# Autodesk Inventor assembly: still pipe
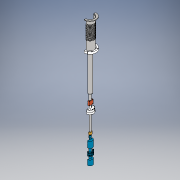
[picture p0: Inventor's stored thumbnail of the model, 180x180]
Saved by Autodesk Inventor 2018 (Build 220112000, 112)
## iProperties
Created: 2019-01-14
Part Number: still pipe
Document SubType Name: Assembly
Designer: Admin
Author: Admin
## Documents named in this file (11)
- C:\Users\Admin\Documents\Cryostat\CAD\still pipe.iam
- C:\Users\Admin\Documents\Cryostat\CAD\KF50 bellows.ipt
- C:\Users\Admin\Documents\Cryostat\CAD\universal connector.ipt
- C:\Users\Admin\Documents\Cryostat\CAD\1in ss pipe.ipt
- C:\Users\Admin\Documents\Cryostat\CAD\adapter.ipt
- C:\Users\Admin\Documents\Cryostat\CAD\heatsink.ipt
- C:\Users\Admin\Documents\Cryostat\CAD\brassbushing2.ipt
- C:\Users\Admin\Documents\Cryostat\CAD\minifridge.ipt
- C:\Users\Admin\Documents\Cryostat\CAD\universal connector male.ipt
- C:\Users\Admin\Documents\Cryostat\CAD\ss pipe for still.ipt
- C:\Users\Admin\Documents\Cryostat\CAD\fridge bushing.ipt
## Components (10 placed, 10 different names)
1. KF50 bellows:1 — Mate:16, Flush:2
2. universal connector:1 — Mate:24, Mate:26, Mate:27, Mate:28, Mate:36
3. 1in ss pipe:3 — Mate:15, Flush:1, Mate:17, Mate:31, Mate:32
4. adapter:1 — Mate:15, Flush:1, Mate:16, Flush:2, Mate:19, Mate:34, Mate:35
5. heatsink:1 — Mate:17, Mate:19, Mate:34, Mate:35
6. brassbushing2:1 — Mate:24, Mate:31, Mate:32, Mate:36
7. minifridge:1 — Mate:41, Mate:42
8. universal connector male:1 — Mate:26, Mate:27, Mate:28, Mate:37, Mate:38
9. ss pipe for still:1 — Mate:37, Mate:38, Mate:39, Mate:40
10. fridge bushing:1 — Mate:39, Mate:40, Mate:41, Mate:42
## Relationships (21: Mate 19, Flush 2)
- Mate:15: 1in ss pipe:3 ↔ adapter:1
- Flush:1: 1in ss pipe:3 ↔ adapter:1
- Mate:16: KF50 bellows:1 ↔ adapter:1
- Flush:2: KF50 bellows:1 ↔ adapter:1
- Mate:17: 1in ss pipe:3 ↔ heatsink:1
- Mate:19: adapter:1 ↔ heatsink:1
- Mate:24: universal connector:1 ↔ brassbushing2:1
- Mate:26: universal connector:1 ↔ universal connector male:1
- Mate:27: universal connector:1 ↔ universal connector male:1
- Mate:28: universal connector:1 ↔ universal connector male:1
- Mate:31: 1in ss pipe:3 ↔ brassbushing2:1
- Mate:32: 1in ss pipe:3 ↔ brassbushing2:1
- Mate:34: adapter:1 ↔ heatsink:1
- Mate:35: adapter:1 ↔ heatsink:1
- Mate:36: universal connector:1 ↔ brassbushing2:1
- Mate:37: universal connector male:1 ↔ ss pipe for still:1
- Mate:38: universal connector male:1 ↔ ss pipe for still:1
- Mate:39: ss pipe for still:1 ↔ fridge bushing:1
- Mate:40: ss pipe for still:1 ↔ fridge bushing:1
- Mate:41: minifridge:1 ↔ fridge bushing:1
- Mate:42: minifridge:1 ↔ fridge bushing:1
